# Autodesk Inventor assembly: setup_full_20260127_RK_4_with_webcams_JF_2
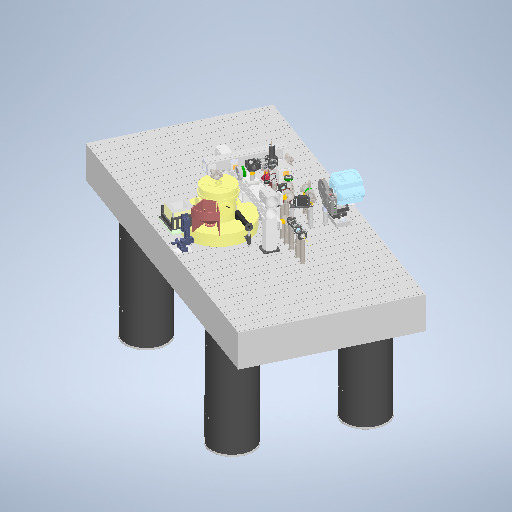
[picture p0: Inventor's stored thumbnail of the model, 512x512]
Saved by Autodesk Inventor 2026.1 (Build 301233000, 233)
## iProperties
Created: 2018-05-08
Part Number: setup_full_20260127_RK_4_with_webcams_JF_2
Document SubType Name: Assembly
Designer: rainer
Author: rainer
## Documents named in this file (45)
- C:\Users\user\Desktop\setup for publishing\setup_full_20260127_RK_4_with_webcams_JF_2.iam
- C:\Users\user\Desktop\setup for publishing\table.ipt
- C:\Users\user\Desktop\setup for publishing\CF9512_mounting_lugs.ipt
- C:\Users\user\Desktop\setup for publishing\base_assembly.iam
- C:\Users\user\Desktop\setup for publishing\Liftinglug.ipt
- C:\Users\user\Desktop\setup for publishing\RM_8010_M_50(Magnetic Piston,0,B,0).iam
- C:\Users\user\Desktop\setup for publishing\Bolzen.ipt
- C:\Users\user\Desktop\setup for publishing\Verbinder_Tisch_Dewar_gespiegelt.ipt
- C:\Users\user\Desktop\setup for publishing\Verbinder_Tisch_Dewar_alt.ipt
- C:\Users\user\Desktop\setup for publishing\kinematic-mount-assembly.iam
- C:\Users\user\Desktop\setup for publishing\Insulation_4.ipt
- C:\Users\user\Desktop\setup for publishing\attocube_stack_ohne_heater_ohne_boden.iam
- C:\Users\user\Desktop\setup for publishing\Camera+Adapter+Filterwheel+Poles.iam
- C:\Users\user\Desktop\setup for publishing\bridge_final.iam
- C:\Users\user\Desktop\setup for publishing\6inch_mirror.iam
- C:\Users\user\Desktop\setup for publishing\insulation_lid_objective.ipt
- C:\Users\user\Desktop\setup for publishing\insulation_lid_objective_adapter.ipt
- C:\Users\user\Desktop\setup for publishing\sample-transfer.iam
- C:\Users\user\Desktop\setup for publishing\160mmLens_assembly_table.iam
- C:\Users\user\Desktop\setup for publishing\sample-transferbox.ipt
- C:\Users\user\Desktop\setup for publishing\XYZ.iam
- C:\Users\user\Desktop\setup for publishing\complete mount for leica brick.iam
- C:\Users\user\Desktop\setup for publishing\Becher gegen Wind.ipt
- C:\Users\user\Desktop\setup for publishing\inner_gas_outlet_v2_2020.ipt
- C:\Users\user\Desktop\setup for publishing\lamellen_2020.ipt
- C:\Users\user\Desktop\setup for publishing\a new funnel_ again.ipt
- C:\Users\user\Desktop\setup for publishing\N2-vent.iam
- C:\Users\user\Desktop\setup for publishing\Laser.iam
- C:\Users\user\Desktop\setup for publishing\slider for beam diameter.iam
- C:\Users\user\Desktop\setup for publishing\circular polarizer.iam
- C:\Users\user\Desktop\setup for publishing\slider for Reflection.iam
- C:\Users\user\Desktop\setup for publishing\LED mount and arm.iam
- C:\Users\user\Desktop\setup for publishing\Norhof wire channel top.ipt
- C:\Users\user\Desktop\setup for publishing\Kabelstopfen_Hinten_next try.ipt
- C:\Users\user\Desktop\setup for publishing\heater plug.ipt
- C:\Users\user\Desktop\setup for publishing\stopfen hinten.ipt
- C:\Users\user\Desktop\setup for publishing\moto filter whel.iam
- C:\Users\user\Desktop\setup for publishing\LeicTransfer Halter.ipt
- C:\Users\user\Desktop\setup for publishing\deformable mirror.iam
- C:\Users\user\Desktop\setup for publishing\stopfen-front.ipt
- C:\Users\user\Desktop\setup for publishing\Isolierung_StopfenLinksRechts_rk.ipt
- C:\Users\user\Desktop\setup for publishing\webcam_new.ipt
- C:\Users\user\Desktop\setup for publishing\Isolierung_StopfenLinksRechts_rk._linksJF.ipt
- C:\Users\user\Desktop\setup for publishing\T1020CK-Step_feetOnly.iam
- N:\Projects\setup\backup_inventor and 3D-Print\inventor\setup_full_20201005.iam
## Components (52 placed, 43 different names)
1. table:1 — Passend:40, Passend:41, Passend:45, Fluchtend:6, Passend:46, Winkel:1, Passend:77, Passend:78, Passend:111, Passend:114, Passend:115, Passend:153, Passend:155, Passend:175, Passend:180, Winkel:2, Passend:209, Passend:210, Winkel:3, Passend:238, Passend:240, Passend:243, Passend:246, Winkel:5, Winkel:6, Winkel:7, Winkel:9, Passend:267, Passend:268, Passend:270, Passend:271, Passend:274, Passend:308, Tangential:1, Tangential:2, Tangential:3
2. T1020CK-Step_feetOnly:1 [sub-assembly] — Passend:308, Tangential:1, Tangential:2, Tangential:3
3. Dewar with lifting lugs — Passend:21, Passend:22, Fluchtend:1, Fluchtend:2, Passend:23, Fluchtend:3, Fluchtend:4, Passend:24, Fluchtend:5, Passend:45, Fluchtend:6
4. Liftinglug:1 — Passend:21, Passend:22, Fluchtend:1
5. Liftinglug:2 — Fluchtend:2, Passend:23, Fluchtend:3
6. Liftinglug:3 — Fluchtend:4, Passend:24, Fluchtend:5
7. Verbinder_Tisch_Dewar_gespiegelt:1 — Passend:33, Passend:34, Passend:40, Passend:180, Winkel:6, Passend:263
8. Verbinder_Tisch_Dewar_gespiegelt:2 — Passend:41, Passend:175, Winkel:7, Passend:282, Passend:283, Winkel:12
9. Verbinder_Tisch_Dewar_alt:1 — Passend:77, Passend:78, Winkel:5, Passend:280, Passend:281, Winkel:11
10. RM_8010_M_50(Magnetic Piston,0,B,0):1 [sub-assembly] — Passend:33, Passend:34, Passend:307
11. RM_8010_M_50(Magnetic Piston,0,B,0):2 [sub-assembly] — Passend:282, Passend:283, Winkel:12, Passend:284, Passend:285
12. RM_8010_M_50(Magnetic Piston,0,B,0):3 [sub-assembly] — Passend:280, Passend:281, Winkel:11, Passend:286, Passend:287
13. Bolzen:4 — Passend:286, Passend:287
14. Bolzen:5 — Passend:284, Passend:285
15. Bolzen:3 — Passend:263, Passend:307
16. Insulation_4:1 — Passend:72, Passend:73, Passend:74, Passend:111, Passend:122, Passend:234, Passend:235, Passend:253, Passend:254, Passend:255, Passend:256, Passend:257, Passend:258, Passend:259, Passend:260, Passend:295, Passend:300
17. insulation_lid_objective:1 — Passend:122, Passend:123, Winkel:9
18. insulation_lid_objective_adapter:1 — Passend:124, Passend:125
19. Isolierung_StopfenLinksRechts_rk:1 — Passend:299, Passend:300, Winkel:13, Passend:303, Fluchtend:172
20. Isolierung_StopfenLinksRechts_rk._linksJF:1 — Passend:304, Passend:305, Passend:306, Fluchtend:173, Winkel:14
21. webcam_new:2 — Passend:306, Fluchtend:173
22. webcam_new:1 — Passend:303, Fluchtend:172
23. stopfen-front:1 — Passend:295, Passend:296
24. stopfen hinten:1 — Passend:259, Passend:260
25. heater plug:1 — Passend:257, Passend:258
26. Kabelstopfen_Hinten_next try:1 — Passend:255, Passend:256
27. Norhof wire channel top:1 — Passend:253, Passend:254
28. sample-transfer:1 [sub-assembly] — Passend:172, Passend:173, Passend:174, Passend:195, Passend:198, Passend:296
29. a new funnel_ again:1 — Passend:234, Passend:235, Winkel:3
30. N2-vent:2 [sub-assembly] — Winkel:15
31. base_assembly:1 [sub-assembly] — Passend:46, Winkel:1, Passend:69, Passend:70, Passend:71, Passend:72, Passend:73, Passend:74, Passend:79, Passend:80, Passend:81, Fluchtend:151, Passend:171, Passend:172, Passend:173, Passend:174, Passend:214, Passend:215, Passend:216, Passend:217, Passend:218, Passend:219, Passend:220, Passend:221, Passend:222, Passend:299, Passend:304, Passend:305
32. attocube_stack_ohne_heater_ohne_boden:1 [sub-assembly] — Passend:79, Passend:80, Passend:81, Passend:211, Passend:212, Passend:213
33. Becher gegen Wind:1 — Passend:214, Passend:215, Passend:216
34. inner_gas_outlet_v2_2020:1 — Passend:217, Passend:218, Passend:219
35. lamellen_2020:1 — Passend:220, Passend:221, Passend:222
36. complete mount for leica brick:1 [sub-assembly] — Passend:211, Passend:212, Passend:213
37. kinematic-mount-assembly:1 [sub-assembly] — Passend:69, Passend:70, Passend:71, Passend:123, Passend:124, Passend:125, Passend:154
38. bridge_final:1 [sub-assembly] — Passend:114, Passend:115, Passend:153, Passend:154, Passend:155, Passend:239, Fluchtend:166, Passend:241, Passend:242, Passend:244, Passend:245, Passend:247, Passend:248, Passend:249, Passend:250, Passend:288, Passend:289, Winkel:13, Winkel:15
39. sample-transferbox:1 — Passend:195, Winkel:2, Passend:198, Passend:264
40. Camera+Adapter+Filterwheel+Poles:2 [sub-assembly] — Passend:274, Passend:278, Winkel:10, Passend:279, Fluchtend:170, Fluchtend:171
41. moto filter whel:2 [sub-assembly] — Passend:278, Winkel:10, Passend:279
42. XYZ:1 [sub-assembly] — Passend:209, Passend:210, Passend:264, Passend:265, Passend:266, Winkel:8
43. LeicTransfer Halter:1 — Passend:265, Passend:266, Winkel:8
44. Laser:1 [sub-assembly] — Passend:238, Passend:239, Fluchtend:166
45. slider for beam diameter:1 [sub-assembly] — Passend:240, Passend:241, Passend:242
46. circular polarizer:1 [sub-assembly] — Passend:243, Passend:244, Passend:245
47. slider for Reflection:1 [sub-assembly] — Passend:246, Passend:247, Passend:248, Passend:251
48. LED mount and arm:1 [sub-assembly] — Passend:249, Passend:250, Passend:251
49. deformable mirror:1 [sub-assembly] — Passend:267, Passend:288, Passend:289, Passend:290, Passend:291
50. 6inch_mirror:3 [sub-assembly] — Passend:268, Passend:290, Passend:291, Passend:292, Passend:293
51. 160mmLens_assembly_table:2 [sub-assembly] — Passend:270, Passend:292, Passend:293, Fluchtend:169, Passend:294
52. 6inch_mirror:4 [sub-assembly] — Passend:271, Fluchtend:169, Passend:294, Fluchtend:170, Fluchtend:171
## Relationships (145: Mate 115, Angle 14, Flush 13, Tangent 3)
- Passend:21 [Mate]: Dewar with lifting lugs ↔ Liftinglug:1
- Passend:22 [Mate]: Dewar with lifting lugs ↔ Liftinglug:1
- Fluchtend:1 [Flush]: Dewar with lifting lugs ↔ Liftinglug:1
- Fluchtend:2 [Flush]: Dewar with lifting lugs ↔ Liftinglug:2
- Passend:23 [Mate]: Dewar with lifting lugs ↔ Liftinglug:2
- Fluchtend:3 [Flush]: Dewar with lifting lugs ↔ Liftinglug:2
- Fluchtend:4 [Flush]: Dewar with lifting lugs ↔ Liftinglug:3
- Passend:24 [Mate]: Dewar with lifting lugs ↔ Liftinglug:3
- Fluchtend:5 [Flush]: Dewar with lifting lugs ↔ Liftinglug:3
- Passend:33 [Mate] (0.5 mm): Verbinder_Tisch_Dewar_gespiegelt:1 ↔ RM_8010_M_50(Magnetic Piston,0,B,0):1
- Passend:34 [Mate] (0.5 mm): Verbinder_Tisch_Dewar_gespiegelt:1 ↔ RM_8010_M_50(Magnetic Piston,0,B,0):1
- Passend:40 [Mate]: table:1 ↔ Verbinder_Tisch_Dewar_gespiegelt:1
- Passend:41 [Mate]: table:1 ↔ Verbinder_Tisch_Dewar_gespiegelt:2
- Passend:45 [Mate]: table:1 ↔ Dewar with lifting lugs
- Fluchtend:6 [Flush]: table:1 ↔ Dewar with lifting lugs
- Passend:46 [Mate]: table:1 ↔ base_assembly:1
- Winkel:1 [Angle] (0 deg): table:1 ↔ base_assembly:1
- Passend:69 [Mate]: base_assembly:1 ↔ kinematic-mount-assembly:1
- Passend:70 [Mate]: base_assembly:1 ↔ kinematic-mount-assembly:1
- Passend:71 [Mate]: base_assembly:1 ↔ kinematic-mount-assembly:1
- Passend:72 [Mate]: Insulation_4:1 ↔ base_assembly:1
- Passend:73 [Mate]: Insulation_4:1 ↔ base_assembly:1
- Passend:74 [Mate]: Insulation_4:1 ↔ base_assembly:1
- Passend:77 [Mate]: table:1 ↔ Verbinder_Tisch_Dewar_alt:1
- Passend:78 [Mate]: table:1 ↔ Verbinder_Tisch_Dewar_alt:1
- Passend:79 [Mate]: base_assembly:1 ↔ attocube_stack_ohne_heater_ohne_boden:1
- Passend:80 [Mate]: base_assembly:1 ↔ attocube_stack_ohne_heater_ohne_boden:1
- Passend:81 [Mate]: base_assembly:1 ↔ attocube_stack_ohne_heater_ohne_boden:1
- Passend:111 [Mate]: table:1 ↔ Insulation_4:1
- Passend:114 [Mate]: table:1 ↔ bridge_final:1
- Passend:115 [Mate]: table:1 ↔ bridge_final:1
- Passend:122 [Mate]: Insulation_4:1 ↔ insulation_lid_objective:1
- Passend:123 [Mate]: insulation_lid_objective:1 ↔ kinematic-mount-assembly:1
- Passend:124 [Mate]: insulation_lid_objective_adapter:1 ↔ kinematic-mount-assembly:1
- Passend:125 [Mate]: insulation_lid_objective_adapter:1 ↔ kinematic-mount-assembly:1
- Passend:153 [Mate]: table:1 ↔ bridge_final:1
- Passend:154 [Mate]: kinematic-mount-assembly:1 ↔ bridge_final:1
- Passend:155 [Mate]: table:1 ↔ bridge_final:1
- Fluchtend:151 [Flush] (25 mm): base_assembly:1
- Passend:171 [Mate]: base_assembly:1
- Passend:172 [Mate]: sample-transfer:1 ↔ base_assembly:1
- Passend:173 [Mate]: sample-transfer:1 ↔ base_assembly:1
- Passend:174 [Mate]: sample-transfer:1 ↔ base_assembly:1
- Passend:175 [Mate]: table:1 ↔ Verbinder_Tisch_Dewar_gespiegelt:2
- Passend:180 [Mate]: table:1 ↔ Verbinder_Tisch_Dewar_gespiegelt:1
- Passend:195 [Mate]: sample-transfer:1 ↔ sample-transferbox:1
- Winkel:2 [Angle] (0 deg): table:1 ↔ sample-transferbox:1
- Passend:198 [Mate]: sample-transfer:1 ↔ sample-transferbox:1
- Passend:209 [Mate]: table:1 ↔ XYZ:1
- Passend:210 [Mate]: table:1 ↔ XYZ:1
- Passend:211 [Mate]: attocube_stack_ohne_heater_ohne_boden:1 ↔ complete mount for leica brick:1
- Passend:212 [Mate]: attocube_stack_ohne_heater_ohne_boden:1 ↔ complete mount for leica brick:1
- Passend:213 [Mate]: attocube_stack_ohne_heater_ohne_boden:1 ↔ complete mount for leica brick:1
- Passend:214 [Mate]: base_assembly:1 ↔ Becher gegen Wind:1
- Passend:215 [Mate]: base_assembly:1 ↔ Becher gegen Wind:1
- Passend:216 [Mate]: base_assembly:1 ↔ Becher gegen Wind:1
- Passend:217 [Mate]: base_assembly:1 ↔ inner_gas_outlet_v2_2020:1
- Passend:218 [Mate]: base_assembly:1 ↔ inner_gas_outlet_v2_2020:1
- Passend:219 [Mate]: base_assembly:1 ↔ inner_gas_outlet_v2_2020:1
- Passend:220 [Mate]: base_assembly:1 ↔ lamellen_2020:1
- Passend:221 [Mate]: base_assembly:1 ↔ lamellen_2020:1
- Passend:222 [Mate]: base_assembly:1 ↔ lamellen_2020:1
- Passend:234 [Mate]: Insulation_4:1 ↔ a new funnel_ again:1
- Passend:235 [Mate]: Insulation_4:1 ↔ a new funnel_ again:1
- Winkel:3 [Angle] (145 deg): table:1 ↔ a new funnel_ again:1
- [Mate]: table:1 ↔ N2-vent:2
- [Mate]: Insulation_4:1 ↔ N2-vent:2
- Passend:238 [Mate]: table:1 ↔ Laser:1
- Passend:239 [Mate]: bridge_final:1 ↔ Laser:1
- Fluchtend:166 [Flush] (90 mm): bridge_final:1 ↔ Laser:1
- Passend:240 [Mate]: table:1 ↔ slider for beam diameter:1
- Passend:241 [Mate] (335 mm): bridge_final:1 ↔ slider for beam diameter:1
- Passend:242 [Mate] (49 mm): bridge_final:1 ↔ slider for beam diameter:1
- Passend:243 [Mate]: table:1 ↔ circular polarizer:1
- Passend:244 [Mate] (70 mm): bridge_final:1 ↔ circular polarizer:1
- Passend:245 [Mate] (51 mm): bridge_final:1 ↔ circular polarizer:1
- Passend:246 [Mate]: table:1 ↔ slider for Reflection:1
- Passend:247 [Mate] (80 mm): bridge_final:1 ↔ slider for Reflection:1
- Passend:248 [Mate] (19 mm): bridge_final:1 ↔ slider for Reflection:1
- Passend:249 [Mate]: bridge_final:1 ↔ LED mount and arm:1
- Passend:250 [Mate]: bridge_final:1 ↔ LED mount and arm:1
- Passend:251 [Mate]: slider for Reflection:1 ↔ LED mount and arm:1
- Passend:253 [Mate]: Insulation_4:1 ↔ Norhof wire channel top:1
- Passend:254 [Mate]: Insulation_4:1 ↔ Norhof wire channel top:1
- Passend:255 [Mate]: Insulation_4:1 ↔ Kabelstopfen_Hinten_next try:1
- Passend:256 [Mate] (90 mm): Insulation_4:1 ↔ Kabelstopfen_Hinten_next try:1
- Passend:257 [Mate]: Insulation_4:1 ↔ heater plug:1
- Passend:258 [Mate]: Insulation_4:1 ↔ heater plug:1
- Passend:259 [Mate]: Insulation_4:1 ↔ stopfen hinten:1
- Passend:260 [Mate]: Insulation_4:1 ↔ stopfen hinten:1
- Winkel:5 [Angle] (0 deg): table:1 ↔ Verbinder_Tisch_Dewar_alt:1
- Winkel:6 [Angle] (180 deg): table:1 ↔ Verbinder_Tisch_Dewar_gespiegelt:1
- Winkel:7 [Angle] (0 deg): table:1 ↔ Verbinder_Tisch_Dewar_gespiegelt:2
- Passend:263 [Mate]: Verbinder_Tisch_Dewar_gespiegelt:1 ↔ Bolzen:3
- Passend:264 [Mate]: sample-transferbox:1 ↔ XYZ:1
- Passend:265 [Mate]: XYZ:1 ↔ LeicTransfer Halter:1
- Passend:266 [Mate]: XYZ:1 ↔ LeicTransfer Halter:1
- Winkel:8 [Angle] (0 deg): XYZ:1 ↔ LeicTransfer Halter:1
- Winkel:9 [Angle] (-130 deg): table:1 ↔ insulation_lid_objective:1
- Passend:267 [Mate]: table:1 ↔ deformable mirror:1
- Passend:268 [Mate]: table:1 ↔ 6inch_mirror:3
- Passend:270 [Mate]: table:1 ↔ 160mmLens_assembly_table:2
- Passend:271 [Mate]: table:1 ↔ 6inch_mirror:4
- Passend:274 [Mate]: table:1 ↔ Camera+Adapter+Filterwheel+Poles:2
- Passend:278 [Mate]: Camera+Adapter+Filterwheel+Poles:2 ↔ moto filter whel:2
- Winkel:10 [Angle] (180 deg): Camera+Adapter+Filterwheel+Poles:2 ↔ moto filter whel:2
- Passend:279 [Mate]: Camera+Adapter+Filterwheel+Poles:2 ↔ moto filter whel:2
- Passend:280 [Mate]: Verbinder_Tisch_Dewar_alt:1 ↔ RM_8010_M_50(Magnetic Piston,0,B,0):3
- Passend:281 [Mate]: Verbinder_Tisch_Dewar_alt:1 ↔ RM_8010_M_50(Magnetic Piston,0,B,0):3
- Winkel:11 [Angle] (0 deg): Verbinder_Tisch_Dewar_alt:1 ↔ RM_8010_M_50(Magnetic Piston,0,B,0):3
- Passend:282 [Mate]: Verbinder_Tisch_Dewar_gespiegelt:2 ↔ RM_8010_M_50(Magnetic Piston,0,B,0):2
- Passend:283 [Mate]: Verbinder_Tisch_Dewar_gespiegelt:2 ↔ RM_8010_M_50(Magnetic Piston,0,B,0):2
- Winkel:12 [Angle] (0 deg): Verbinder_Tisch_Dewar_gespiegelt:2 ↔ RM_8010_M_50(Magnetic Piston,0,B,0):2
- Passend:284 [Mate]: RM_8010_M_50(Magnetic Piston,0,B,0):2 ↔ Bolzen:5
- Passend:285 [Mate]: RM_8010_M_50(Magnetic Piston,0,B,0):2 ↔ Bolzen:5
- Passend:286 [Mate]: RM_8010_M_50(Magnetic Piston,0,B,0):3 ↔ Bolzen:4
- Passend:287 [Mate]: RM_8010_M_50(Magnetic Piston,0,B,0):3 ↔ Bolzen:4
- Passend:288 [Mate]: bridge_final:1 ↔ deformable mirror:1
- Passend:289 [Mate] (210 mm): bridge_final:1 ↔ deformable mirror:1
- Passend:290 [Mate]: deformable mirror:1 ↔ 6inch_mirror:3
- Passend:291 [Mate] (120 mm): deformable mirror:1 ↔ 6inch_mirror:3
- Passend:292 [Mate]: 6inch_mirror:3 ↔ 160mmLens_assembly_table:2
- Passend:293 [Mate] (39 mm): 6inch_mirror:3 ↔ 160mmLens_assembly_table:2
- Fluchtend:169 [Flush]: 160mmLens_assembly_table:2 ↔ 6inch_mirror:4
- Passend:294 [Mate] (23 mm): 160mmLens_assembly_table:2 ↔ 6inch_mirror:4
- Fluchtend:170 [Flush]: Camera+Adapter+Filterwheel+Poles:2 ↔ 6inch_mirror:4
- Fluchtend:171 [Flush] (110 mm): Camera+Adapter+Filterwheel+Poles:2 ↔ 6inch_mirror:4
- Passend:295 [Mate]: Insulation_4:1 ↔ stopfen-front:1
- Passend:296 [Mate]: stopfen-front:1 ↔ sample-transfer:1
- Passend:299 [Mate] (5 mm): Isolierung_StopfenLinksRechts_rk:1 ↔ base_assembly:1
- Passend:300 [Mate]: Insulation_4:1 ↔ Isolierung_StopfenLinksRechts_rk:1
- Winkel:13 [Angle] (0 deg): Isolierung_StopfenLinksRechts_rk:1 ↔ bridge_final:1
- Passend:303 [Mate]: Isolierung_StopfenLinksRechts_rk:1 ↔ webcam_new:1
- Fluchtend:172 [Flush]: Isolierung_StopfenLinksRechts_rk:1 ↔ webcam_new:1
- Passend:304 [Mate]: Isolierung_StopfenLinksRechts_rk._linksJF:1 ↔ base_assembly:1
- Passend:305 [Mate] (5 mm): Isolierung_StopfenLinksRechts_rk._linksJF:1 ↔ base_assembly:1
- Passend:306 [Mate]: Isolierung_StopfenLinksRechts_rk._linksJF:1 ↔ webcam_new:2
- Fluchtend:173 [Flush]: Isolierung_StopfenLinksRechts_rk._linksJF:1 ↔ webcam_new:2
- Winkel:14 [Angle] (125 deg): Isolierung_StopfenLinksRechts_rk._linksJF:1
- Passend:307 [Mate]: RM_8010_M_50(Magnetic Piston,0,B,0):1 ↔ Bolzen:3
- Winkel:15 [Angle] (0 deg): N2-vent:2 ↔ bridge_final:1
- Passend:308 [Mate]: table:1 ↔ T1020CK-Step_feetOnly:1
- Tangential:1 (8.5 mm): table:1 ↔ T1020CK-Step_feetOnly:1
- Tangential:2 (301 mm): table:1 ↔ T1020CK-Step_feetOnly:1
- Tangential:3 (8.5 mm): table:1 ↔ T1020CK-Step_feetOnly:1
